# Autodesk Inventor assembly: modular HDzero micro mount
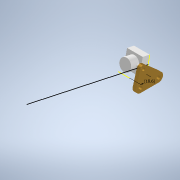
[picture p0: Inventor's stored thumbnail of the model, 180x180]
Saved by Autodesk Inventor 2020 (Build 240168000, 168)
## iProperties
Created: 2022-05-06
Part Number: modular HDzero micro mount
Document SubType Name: Assembly
Designer: Steven
Author: Steven
## Documents named in this file (3)
- Y:\FPV drone stuff\0 Street League\Frames\PB-Kauri-X\3D prints\35 mm canopy\work in progress prints\modular HDzero micro mount.iam
- Y:\FPV drone stuff\0 Street League\Frames\PB-Kauri-X\3D prints\35 mm canopy\work in progress prints\HDzero micro dummy.ipt
- Y:\FPV drone stuff\0 Street League\Frames\PB-Kauri-X\3D prints\35 mm canopy\work in progress prints\Kauri modular camera mount HDzero micro v1.ipt
## Components (2 placed, 2 different names)
1. HDzero micro dummy:1 — Insert:1, Insert:2
2. Kauri modular camera mount HDzero micro v1:1 — Mate:1, Mate:2, Tangent:1, Insert:1, Insert:2
## Relationships (5: Mate 2, Insert 2, Tangent 1)
- Mate:1: Kauri modular camera mount HDzero micro v1:1
- Mate:2: Kauri modular camera mount HDzero micro v1:1
- Tangent:1: Kauri modular camera mount HDzero micro v1:1
- Insert:1: HDzero micro dummy:1 ↔ Kauri modular camera mount HDzero micro v1:1
- Insert:2: HDzero micro dummy:1 ↔ Kauri modular camera mount HDzero micro v1:1
